# Autodesk Inventor assembly: main
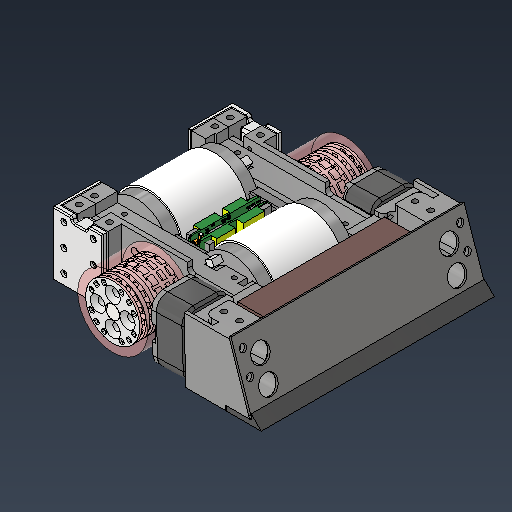
[picture p0: Inventor's stored thumbnail of the model, 512x512]
Saved by Autodesk Inventor 2026.2 (Build 302298010, 298A)
## iProperties
Created: 2026-03-09
Part Number: main
Document SubType Name: Assembly
Designer: szymo
Mass: 796.283 g
Surface Area: 1662.82 cm^2
Volume: 202.049 cm^3
Density: 3.94104 g/cm^3
Author: szymo
## Documents named in this file (24)
- D:\tech\robotyka\robots\evangelion-turbo\inventor-project\main.iam
- D:\tech\robotyka\robots\evangelion-turbo\inventor-project\drive-train.iam
- D:\tech\robotyka\robots\evangelion-turbo\inventor-project\LUNA.ipt
- D:\tech\robotyka\robots\evangelion-turbo\inventor-project\3s450mah.ipt
- D:\tech\robotyka\robots\evangelion-turbo\inventor-project\KTIR-Board.ipt
- D:\tech\robotyka\robots\evangelion-turbo\inventor-project\plug.ipt
- D:\tech\robotyka\robots\evangelion-turbo\inventor-project\FonrtMount.ipt
- D:\tech\robotyka\robots\evangelion-turbo\inventor-project\SteelFront.ipt
- D:\tech\robotyka\robots\evangelion-turbo\inventor-project\SpringSteelFront.ipt
- D:\tech\robotyka\robots\evangelion-turbo\inventor-project\LeftGearbox.ipt
- D:\tech\robotyka\robots\evangelion-turbo\inventor-project\LeftGearboxCoverr.ipt
- D:\tech\robotyka\robots\evangelion-turbo\inventor-project\RightGearbox.ipt
- D:\tech\robotyka\robots\evangelion-turbo\inventor-project\RightGearboxCover.ipt
- D:\tech\robotyka\robots\evangelion-turbo\inventor-project\GearboxBearingHolderCover.ipt
- D:\tech\robotyka\robots\evangelion-turbo\inventor-project\PCBs_Holder.ipt
- D:\tech\robotyka\robots\evangelion-turbo\inventor-project\GearboxBearingHolderCover_MIR.ipt
- D:\tech\robotyka\robots\evangelion-turbo\inventor-project\1703 Fan asm\1703 Fan asm\1703 Fan asm.ipt
- D:\tech\robotyka\robots\evangelion-turbo\inventor-project\LunasCover.ipt
- D:\tech\robotyka\robots\evangelion-turbo\inventor-project\MetalBack.ipt
- D:\tech\robotyka\robots\evangelion-turbo\inventor-project\PCB_Motors\PCB_Motors\PCB_Motors.ipt
- D:\tech\robotyka\robots\evangelion-turbo\inventor-project\Interface_assembly.iam
- D:\tech\robotyka\robots\evangelion-turbo\inventor-project\ceil.ipt
- D:\tech\robotyka\robots\evangelion-turbo\inventor-project\BackLunaRecoveryHold.ipt
- D:\tech\robotyka\robots\evangelion-turbo\inventor-project\BackLunaRecoveryHold_MIR.ipt
## Components (31 placed, 23 different names)
1. drive-train:1 [sub-assembly] — Flush:2, Flush:3, Flush:4, Mate:2, Mate:3, Tangent:1, Mate:18, Mate:23, Mate:19
2. 3s450mah:1 — Flush:8, Tangent:1, Flush:9
3. ceil:1 — Flush:86
4. MetalBack:1 — Flush:83
5. BackLunaRecoveryHold:1 — Flush:88
6. BackLunaRecoveryHold_MIR:1 — Flush:89
7. LunasCover:1 — Flush:82
8. LunasCover:2 — Mate:35, Mate:36, Mate:37
9. LUNA:2 — Mate:1, Mate:3, Angle:2, Mate:11, Flush:82
10. LUNA:1 — Flush:5, Mate:2, Angle:1, Mate:12, Mate:35, Mate:36, Mate:37
11. LUNA:3 — Flush:22, Flush:23, Mate:6
12. LUNA:4 — Flush:24, Flush:25, Mate:7
13. KTIR-Board:1 — Flush:10, Flush:11, Flush:13
14. KTIR-Board:2 — Mate:4, Flush:12, Flush:14
15. KTIR-Board:4 — Flush:17, Flush:27, Mate:6, Mate:18
16. KTIR-Board:5 — Flush:28, Flush:29, Mate:7, Mate:19
17. SpringSteelFront:1 — Flush:65, Mate:21, Mate:22
18. SteelFront:1 — Mate:33, Flush:81, Mate:34
19. plug:1 — Mate:10, Flush:87, Mate:20
20. FonrtMount:1 — Flush:47, Mate:33
21. GearboxBearingHolderCover:1 — Flush:74
22. LeftGearbox:1 — Flush:67, Mate:51
23. LeftGearboxCoverr:1 — Flush:69
24. RightGearboxCover:1 — Flush:73, Mate:53
25. RightGearbox:1 — Flush:71, Mate:52, Flush:86
26. GearboxBearingHolderCover_MIR:1 — Mate:23, Flush:78, Flush:79
27. Interface_assembly:1 [sub-assembly] — Mate:51, Mate:52, Mate:53
28. PCB_Motors:1 — Mate:45, Mate:46, Mate:47
29. PCB_Motors:2 — Mate:48, Mate:49, Mate:50
30. 1703 Fan asm:1 — Flush:85, Mate:31, Mate:32
31. PCBs_Holder:1 — Flush:77, Mate:31, Mate:32, Mate:45, Mate:46, Mate:47, Mate:48, Mate:49, Mate:50
## Relationships (76: Flush 42, Mate 31, Angle 2, Tangent 1)
- Flush:2: drive-train:1
- Flush:3 (-19.2 mm): drive-train:1
- Flush:4: drive-train:1
- Flush:5 (50 mm): LUNA:1
- Mate:1 (-50 mm): LUNA:2
- Mate:2 (19 mm): drive-train:1 ↔ LUNA:1
- Mate:3 (19 mm): drive-train:1 ↔ LUNA:2
- Angle:1 (-2 deg): LUNA:1
- Angle:2 (182 deg): LUNA:2
- Flush:8 (4.5 mm): 3s450mah:1
- Tangent:1: drive-train:1 ↔ 3s450mah:1
- Flush:9 (-31.5 mm): 3s450mah:1
- Flush:10 (-46.5 mm): KTIR-Board:1
- Mate:4 (-46.5 mm): KTIR-Board:2
- Flush:11 (0.13 mm): KTIR-Board:1
- Flush:12 (0.13 mm): KTIR-Board:2
- Flush:13 (67 mm): KTIR-Board:1
- Flush:14 (-67 mm): KTIR-Board:2
- Flush:17: KTIR-Board:4
- Flush:22: LUNA:3
- Flush:23 (1 mm): LUNA:3
- Flush:24 (1 mm): LUNA:4
- Flush:25: LUNA:4
- Flush:27 (1 mm): KTIR-Board:4
- Flush:28 (1 mm): KTIR-Board:5
- Flush:29: KTIR-Board:5
- Mate:6 (0.5 mm): LUNA:3 ↔ KTIR-Board:4
- Mate:7 (0.5 mm): LUNA:4 ↔ KTIR-Board:5
- Mate:10: plug:1
- Flush:87: plug:1
- Mate:11: LUNA:2
- Mate:12: LUNA:1
- Flush:47: FonrtMount:1
- Flush:53 (-29 mm)
- Mate:18 (0.5 mm): drive-train:1 ↔ KTIR-Board:4
- Mate:19 (0.5 mm): drive-train:1 ↔ KTIR-Board:5
- Mate:20 (-99 mm): plug:1
- Flush:65: SpringSteelFront:1
- Mate:21: SpringSteelFront:1
- Mate:22: SpringSteelFront:1
- Flush:66 (-19.2 mm)
- Flush:67: LeftGearbox:1
- Flush:68 (-28.5 mm)
- Flush:69: LeftGearboxCoverr:1
- Flush:70 (19.2 mm)
- Flush:71: RightGearbox:1
- Flush:72 (28.5 mm)
- Flush:73: RightGearboxCover:1
- Flush:74: GearboxBearingHolderCover:1
- Flush:77 (1 mm): PCBs_Holder:1
- Mate:23: drive-train:1 ↔ GearboxBearingHolderCover_MIR:1
- Flush:78: GearboxBearingHolderCover_MIR:1
- Flush:79 (3 mm): GearboxBearingHolderCover_MIR:1
- Flush:85: 1703 Fan asm:1
- Mate:31 (0.25 mm): 1703 Fan asm:1 ↔ PCBs_Holder:1
- Mate:32 (0.25 mm): 1703 Fan asm:1 ↔ PCBs_Holder:1
- Mate:33: SteelFront:1 ↔ FonrtMount:1
- Flush:81 (50 mm): SteelFront:1
- Mate:34 (-3.12 mm): SteelFront:1
- Flush:82: LunasCover:1 ↔ LUNA:2
- Mate:35: LunasCover:2 ↔ LUNA:1
- Mate:36: LunasCover:2 ↔ LUNA:1
- Mate:37: LunasCover:2 ↔ LUNA:1
- Flush:83: MetalBack:1
- Mate:45: PCB_Motors:1 ↔ PCBs_Holder:1
- Mate:46: PCB_Motors:1 ↔ PCBs_Holder:1
- Mate:47: PCB_Motors:1 ↔ PCBs_Holder:1
- Mate:48: PCB_Motors:2 ↔ PCBs_Holder:1
- Mate:49: PCB_Motors:2 ↔ PCBs_Holder:1
- Mate:50: PCB_Motors:2 ↔ PCBs_Holder:1
- Mate:51: LeftGearbox:1 ↔ Interface_assembly:1
- Mate:52 (0.2 mm): RightGearbox:1 ↔ Interface_assembly:1
- Mate:53 (0.2 mm): RightGearboxCover:1 ↔ Interface_assembly:1
- Flush:86: ceil:1 ↔ RightGearbox:1
- Flush:88: BackLunaRecoveryHold:1
- Flush:89: BackLunaRecoveryHold_MIR:1
